# Autodesk Inventor assembly: linear_slider
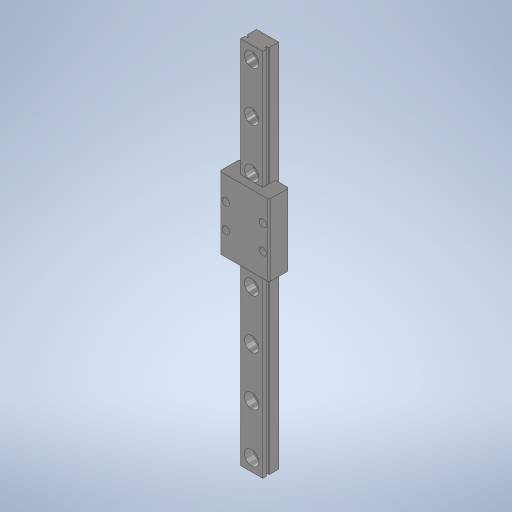
[picture p0: Inventor's stored thumbnail of the model, 512x512]
Saved by Autodesk Inventor 2024 (Build 280153000, 153)
## iProperties
Created: 2025-06-01
Part Number: linear_slider
Document SubType Name: Assembly
Designer: 1412z
Author: 1412z
## Documents named in this file (3)
- C:\Users\1412z\OneDrive\デスクトップ\rdclab\harvesting_robot\harvesting_endeffector\claws_endeffector\linear_actuator\linear_slider.iam
- C:\Users\1412z\OneDrive\デスクトップ\rdclab\harvesting_robot\harvesting_endeffector\claws_endeffector\linear_actuator\rail.ipt
- C:\Users\1412z\OneDrive\デスクトップ\rdclab\harvesting_robot\harvesting_endeffector\claws_endeffector\linear_actuator\slider.ipt
## Components (2 placed, 2 different names)
1. rail:1 — スライダ:1
2. slider:1 — スライダ:1
## Relationships (1: TranslationJoint 1)
- スライダ:1 [TranslationJoint]: rail:1 ↔ slider:1
